# Autodesk Inventor assembly: x_iddler
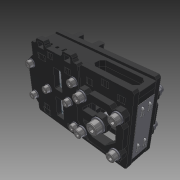
[picture p0: Inventor's stored thumbnail of the model, 180x180]
Saved by Autodesk Inventor 2014 (Build 180170000, 170)
## iProperties
Created: 2014-04-03
Part Number: x_iddler
Document SubType Name: Assembly
Designer: buben
Author: buben
## Documents named in this file (31)
- C:\Users\buben\Documents\GitHub\bacon\inventor files\assemblies\x_iddler.iam
- C:\Users\buben\Documents\GitHub\bacon\inventor files\printer parts\x_iddler_back.ipt
- C:\Users\buben\Documents\GitHub\bacon\inventor files\printer parts\x_motor_smooth_rod_spacer.ipt
- C:\Users\buben\Documents\GitHub\bacon\inventor files\printer parts\x_iddler_wall_upper.ipt
- C:\Users\buben\Documents\GitHub\bacon\inventor files\printer parts\x_iddler_wall_lower.ipt
- C:\Users\buben\Documents\GitHub\bacon\inventor files\printer parts\x_iddler_upper_nut_stop.ipt
- C:\Users\buben\Documents\GitHub\bacon\inventor files\printer parts\x_motor_middle.ipt
- C:\Users\buben\Documents\GitHub\bacon\inventor files\3rd party components\linear_bearing_8\Imported Components\LU8MM\LU8MM.iam
- C:\Users\buben\Documents\GitHub\bacon\inventor files\printer parts\x_motor_top.ipt
- C:\Users\buben\Documents\GitHub\bacon\inventor files\printer parts\x_motor_lower_nut_stop.ipt
- C:\Users\buben\Documents\GitHub\bacon\inventor files\utils\washer_m4.ipt
- C:\Users\buben\Documents\Inventor\Content Center Files\R2014\en-US\ISO 4762(2)\ISO 4762 - M4 x 20ISO.ipt
- C:\Users\buben\Documents\Inventor\Content Center Files\R2014\en-US\ISO 7040\ISO 7040 - M4.ipt
- C:\Users\buben\Documents\Inventor\Content Center Files\R2014\en-US\CSN EN 24032\ISO 4032 - M5CSN EN.ipt
- C:\Users\buben\Documents\GitHub\bacon\inventor files\utils\washer_m5.ipt
- C:\Users\buben\Documents\Inventor\Content Center Files\R2014\en-US\ISO 4762(2)\ISO 4762 - M5 x 50ISO.ipt
- C:\Users\buben\Documents\Inventor\Content Center Files\R2014\en-US\ISO 7040\ISO 7040 - M5.ipt
- C:\Users\buben\Documents\GitHub\bacon\inventor files\printer parts\x_iddler_c_mount.ipt
- C:\Users\buben\Documents\GitHub\bacon\inventor files\printer parts\x_iddler_belt_bearing_mount.ipt
- C:\Users\buben\Documents\GitHub\bacon\inventor files\utils\washer_m6.ipt
- C:\Users\buben\Documents\Inventor\Content Center Files\R2014\en-US\ISO 4762(2)\ISO 4762 - M6 x 60ISO.ipt
- C:\Users\buben\Documents\Inventor\Content Center Files\R2014\en-US\ISO 7040\ISO 7040 - M6.ipt
- C:\Users\buben\Documents\GitHub\bacon\inventor files\utils\washer_m8.ipt
- C:\Users\buben\Documents\Inventor\Content Center Files\R2014\en-US\ISO 7040\ISO 7040 - M8.ipt
- C:\Users\buben\Documents\Inventor\Content Center Files\R2014\en-US\ISO 4762(2)\ISO 4762 - M8 x 65ISO.ipt
- C:\Users\buben\Documents\GitHub\bacon\inventor files\3rd party components\bearing_608\Imported Components\608RS\608RS.ipt
- C:\Users\buben\Documents\GitHub\bacon\inventor files\utils\belt_guide.ipt
- C:\Users\buben\Documents\GitHub\bacon\inventor files\utils\bearing_spacer_1.ipt
- C:\Users\buben\Documents\GitHub\bacon\inventor files\utils\bearing_spacer_2.ipt
- C:\Users\buben\Documents\GitHub\bacon\inventor files\printer parts\x_iddler_right_cap.ipt
- C:\Users\buben\Documents\GitHub\bacon\inventor files\utils\x_iddler_cap_zip_tie.ipt
## Components (80 placed, 30 different names)
1. x_iddler_back:1 — Mate:1, Mate:2, Mate:3, Mate:4, Mate:5, Mate:6, Mate:7, Mate:8, Mate:9, Mate:10, Mate:11, Mate:12, Mate:13, Mate:14, Mate:15, Mate:16, Mate:17, Mate:18, Mate:56, Mate:57, Mate:58, Mate:59, Mate:60, Mate:61, Mate:89, Mate:90, Mate:91, Mate:140
2. x_motor_smooth_rod_spacer:1 — Mate:4, Mate:7, Mate:8
3. x_motor_smooth_rod_spacer:2 — Mate:5, Mate:6, Mate:9
4. x_iddler_wall_upper:1 — Mate:10, Mate:11, Mate:12, Mate:19, Mate:21, Mate:27, Mate:28, Mate:44, Mate:45, Mate:141
5. x_iddler_wall_lower:1 — Mate:13, Mate:14, Mate:15, Mate:20, Flush:1, Mate:30, Mate:31, Mate:32, Mate:33, Mate:34, Mate:35, Mate:47, Mate:48
6. x_iddler_upper_nut_stop:1 — Mate:16, Mate:17, Mate:18, Mate:46, Mate:86, Mate:87, Mate:88
7. x_motor_middle:1 — Mate:19, Mate:20, Mate:21, Mate:22, Mate:23, Mate:24, Mate:26
8. LU8MM:1 [sub-assembly] — Mate:22, Mate:23, Mate:24, Mate:25, Mate:29
9. LU8MM:2 [sub-assembly] — Mate:25, Mate:26
10. x_motor_top:1 — Mate:27, Mate:28, Mate:29, Mate:50, Mate:51, Mate:52, Mate:53, Mate:54, Mate:55, Mate:62, Mate:63, Mate:64, Mate:65, Mate:66, Mate:67
11. x_motor_lower_nut_stop:1 — Flush:1, Mate:30, Mate:31, Mate:36, Mate:38, Mate:49
12. CSN 02 1702 B B 4,3:1 — Mate:36, Mate:37, Mate:40
13. CSN 02 1702 B B 4,3:2 — Mate:38, Mate:39, Mate:42
14. CSN 02 1702 B B 4,3:3 — Mate:33, Mate:34, Insert:2
15. CSN 02 1702 B B 4,3:4 — Mate:32, Mate:35, Insert:1
16. ISO 4762 M4 x 20:1 — Insert:1, Mate:37, Mate:41
17. ISO 4762 M4 x 20:2 — Insert:2, Mate:39, Mate:43
18. DIN EN ISO 7040 M4:1 — Mate:40, Mate:41
19. DIN EN ISO 7040 M4:2 — Mate:42, Mate:43
20. CSN EN 24032 M5:1 — Mate:44, Mate:45, Mate:46
21. CSN EN 24032 M5:2 — Mate:47, Mate:48, Mate:49
22. CSN 02 1702 B B 5,3:1 — Mate:58, Mate:72, Mate:82
23. CSN 02 1702 B B 5,3:2 — Mate:57, Mate:70, Mate:78
24. CSN 02 1702 B B 5,3:3 — Mate:60, Mate:68, Mate:76
25. CSN 02 1702 B B 5,3:4 — Mate:61, Mate:69, Mate:80
26. CSN 02 1702 B B 5,3:5 — Mate:59, Mate:73, Mate:84
27. CSN 02 1702 B B 5,3:6 — Mate:56, Mate:71, Mate:74
28. CSN 02 1702 B B 5,3:7 — Mate:54, Mate:66, Insert:7
29. CSN 02 1702 B B 5,3:8 — Mate:51, Mate:63, Insert:3
30. CSN 02 1702 B B 5,3:9 — Mate:50, Mate:62, Insert:4
31. CSN 02 1702 B B 5,3:10 — Mate:55, Mate:67, Insert:6
32. CSN 02 1702 B B 5,3:11 — Mate:53, Mate:65, Insert:8
33. CSN 02 1702 B B 5,3:12 — Mate:52, Mate:64, Insert:5
34. ISO 4762 M5 x 50:1 — Insert:3, Mate:68, Mate:77
35. ISO 4762 M5 x 50:2 — Insert:4, Mate:69, Mate:81
36. ISO 4762 M5 x 50:3 — Insert:5, Mate:70, Mate:79
37. ISO 4762 M5 x 50:4 — Insert:6, Mate:71, Mate:75
38. ISO 4762 M5 x 50:5 — Insert:7, Mate:72, Mate:83
39. ISO 4762 M5 x 50:6 — Insert:8, Mate:73, Mate:85
40. DIN EN ISO 7040 M5:1 — Mate:78, Mate:79
41. DIN EN ISO 7040 M5:2 — Mate:80, Mate:81
42. DIN EN ISO 7040 M5:3 — Mate:84, Mate:85
43. DIN EN ISO 7040 M5:4 — Mate:82, Mate:83
44. DIN EN ISO 7040 M5:5 — Mate:76, Mate:77
45. DIN EN ISO 7040 M5:6 — Mate:74, Mate:75
46. x_iddler_c_mount:1 — Mate:86, Mate:87, Mate:88, Mate:92, Mate:93, Mate:94
47. x_iddler_belt_bearing_mount:1 — Mate:89, Mate:90, Mate:91, Mate:103, Mate:105, Mate:107, Mate:109, Mate:121, Mate:122, Mate:125, Mate:126
48. x_iddler_belt_bearing_mount:2 — Mate:92, Mate:93, Mate:94, Mate:95, Mate:96, Mate:97, Mate:98, Mate:99, Mate:100, Mate:101, Mate:102, Mate:119, Mate:120, Mate:123, Mate:124
49. CSN 02 1702 B B 6,4:1 — Mate:105, Mate:106, Mate:115
50. CSN 02 1702 B B 6,4:2 — Mate:101, Mate:102, Insert:10
51. CSN 02 1702 B B 6,4:3 — Mate:103, Mate:104, Mate:117
52. CSN 02 1702 B B 6,4:4 — Mate:107, Mate:108, Mate:111
53. CSN 02 1702 B B 6,4:5 — Mate:109, Mate:110, Mate:113
54. CSN 02 1702 B B 6,4:6 — Mate:99, Mate:100, Insert:11
55. CSN 02 1702 B B 6,4:7 — Mate:97, Mate:98, Insert:12
56. CSN 02 1702 B B 6,4:8 — Mate:95, Mate:96, Insert:9
57. ISO 4762 M6 x 60:3 — Insert:9, Mate:110, Mate:114
58. ISO 4762 M6 x 60:4 — Insert:10, Mate:108, Mate:112, Mate:144, Mate:145
59. ISO 4762 M6 x 60:2 — Insert:11, Mate:104, Mate:118, Tangent:1, Mate:142, Mate:143
60. ISO 4762 M6 x 60:1 — Insert:12, Mate:106, Mate:116
61. DIN EN ISO 7040 M6:1 — Mate:115, Mate:116
62. DIN EN ISO 7040 M6:2 — Mate:111, Mate:112
63. DIN EN ISO 7040 M6:3 — Mate:113, Mate:114
64. DIN EN ISO 7040 M6:4 — Mate:117, Mate:118
65. CSN 02 1702 B B 8,4:1 — Mate:119, Mate:120, Insert:13
66. CSN 02 1702 B B 8,4:2 — Mate:121, Mate:122, Mate:127
67. CSN 02 1702 B B 8,4:3 — Mate:123, Mate:124
68. CSN 02 1702 B B 8,4:4 — Mate:125, Mate:126, Mate:136
69. ISO 4762 M8 x 65:1 — Insert:13, Mate:128, Mate:139
70. DIN EN ISO 7040 M8:1 — Mate:127, Mate:128
71. 608RS:1 — Mate:129, Mate:130, Mate:133, Mate:134, Mate:135, Mate:137, Mate:138
72. belt_guide:1 — Mate:129, Mate:130, Mate:131, Mate:132
73. belt_guide:2 — Mate:131, Mate:132, Mate:133
74. bearing_spacer_1:1 — Mate:134, Mate:135, Mate:136
75. bearing_spacer_2:1 — Mate:137, Mate:138, Mate:139
76. x_iddler_right_cap:1 — Mate:140, Mate:141, Tangent:1, Angle:1, Angle:2, Angle:3, Angle:4, Tangent:2, Tangent:3, Tangent:4, Tangent:5
77. x_iddler_cap_zip_tie:1 — Mate:142, Angle:3, Tangent:3
78. x_iddler_cap_zip_tie:2 — Mate:143, Angle:1, Tangent:4
79. x_iddler_cap_zip_tie:3 — Mate:144, Angle:4, Tangent:2
80. x_iddler_cap_zip_tie:4 — Mate:145, Angle:2, Tangent:5
## Relationships (168: Mate 145, Insert 13, Tangent 5, Angle 4, Flush 1)
- Mate:1: x_iddler_back:1
- Mate:2: x_iddler_back:1
- Mate:3: x_iddler_back:1
- Mate:4: x_iddler_back:1 ↔ x_motor_smooth_rod_spacer:1
- Mate:5: x_iddler_back:1 ↔ x_motor_smooth_rod_spacer:2
- Mate:6: x_iddler_back:1 ↔ x_motor_smooth_rod_spacer:2
- Mate:7: x_iddler_back:1 ↔ x_motor_smooth_rod_spacer:1
- Mate:8: x_iddler_back:1 ↔ x_motor_smooth_rod_spacer:1
- Mate:9: x_iddler_back:1 ↔ x_motor_smooth_rod_spacer:2
- Mate:10: x_iddler_back:1 ↔ x_iddler_wall_upper:1
- Mate:11: x_iddler_back:1 ↔ x_iddler_wall_upper:1
- Mate:12: x_iddler_back:1 ↔ x_iddler_wall_upper:1
- Mate:13: x_iddler_back:1 ↔ x_iddler_wall_lower:1
- Mate:14: x_iddler_back:1 ↔ x_iddler_wall_lower:1
- Mate:15: x_iddler_back:1 ↔ x_iddler_wall_lower:1
- Mate:16: x_iddler_back:1 ↔ x_iddler_upper_nut_stop:1
- Mate:17: x_iddler_back:1 ↔ x_iddler_upper_nut_stop:1
- Mate:18: x_iddler_back:1 ↔ x_iddler_upper_nut_stop:1
- Mate:19: x_iddler_wall_upper:1 ↔ x_motor_middle:1
- Mate:20: x_iddler_wall_lower:1 ↔ x_motor_middle:1
- Mate:21: x_iddler_wall_upper:1 ↔ x_motor_middle:1
- Mate:22 (7.5 mm): x_motor_middle:1 ↔ LU8MM:1
- Mate:23 (7.5 mm): x_motor_middle:1 ↔ LU8MM:1
- Mate:24 (0.5 mm): x_motor_middle:1 ↔ LU8MM:1
- Mate:25: LU8MM:1 ↔ LU8MM:2
- Mate:26 (0.5 mm): x_motor_middle:1 ↔ LU8MM:2
- Mate:27: x_iddler_wall_upper:1 ↔ x_motor_top:1
- Mate:28: x_iddler_wall_upper:1 ↔ x_motor_top:1
- Mate:29 (7.5 mm): LU8MM:1 ↔ x_motor_top:1
- Flush:1: x_iddler_wall_lower:1 ↔ x_motor_lower_nut_stop:1
- Mate:30: x_iddler_wall_lower:1 ↔ x_motor_lower_nut_stop:1
- Mate:31: x_iddler_wall_lower:1 ↔ x_motor_lower_nut_stop:1
- Mate:32: x_iddler_wall_lower:1 ↔ CSN 02 1702 B B 4,3:4
- Mate:33: x_iddler_wall_lower:1 ↔ CSN 02 1702 B B 4,3:3
- Mate:34: x_iddler_wall_lower:1 ↔ CSN 02 1702 B B 4,3:3
- Mate:35: x_iddler_wall_lower:1 ↔ CSN 02 1702 B B 4,3:4
- Insert:1: CSN 02 1702 B B 4,3:4 ↔ ISO 4762 M4 x 20:1
- Insert:2: CSN 02 1702 B B 4,3:3 ↔ ISO 4762 M4 x 20:2
- Mate:36: x_motor_lower_nut_stop:1 ↔ CSN 02 1702 B B 4,3:1
- Mate:37: CSN 02 1702 B B 4,3:1 ↔ ISO 4762 M4 x 20:1
- Mate:38: x_motor_lower_nut_stop:1 ↔ CSN 02 1702 B B 4,3:2
- Mate:39: CSN 02 1702 B B 4,3:2 ↔ ISO 4762 M4 x 20:2
- Mate:40: CSN 02 1702 B B 4,3:1 ↔ DIN EN ISO 7040 M4:1
- Mate:41: ISO 4762 M4 x 20:1 ↔ DIN EN ISO 7040 M4:1
- Mate:42: CSN 02 1702 B B 4,3:2 ↔ DIN EN ISO 7040 M4:2
- Mate:43: ISO 4762 M4 x 20:2 ↔ DIN EN ISO 7040 M4:2
- Mate:44: x_iddler_wall_upper:1 ↔ CSN EN 24032 M5:1
- Mate:45: x_iddler_wall_upper:1 ↔ CSN EN 24032 M5:1
- Mate:46: x_iddler_upper_nut_stop:1 ↔ CSN EN 24032 M5:1
- Mate:47: x_iddler_wall_lower:1 ↔ CSN EN 24032 M5:2
- Mate:48: x_iddler_wall_lower:1 ↔ CSN EN 24032 M5:2
- Mate:49: x_motor_lower_nut_stop:1 ↔ CSN EN 24032 M5:2
- Mate:50: x_motor_top:1 ↔ CSN 02 1702 B B 5,3:9
- Mate:51: x_motor_top:1 ↔ CSN 02 1702 B B 5,3:8
- Mate:52: x_motor_top:1 ↔ CSN 02 1702 B B 5,3:12
- Mate:53: x_motor_top:1 ↔ CSN 02 1702 B B 5,3:11
- Mate:54: x_motor_top:1 ↔ CSN 02 1702 B B 5,3:7
- Mate:55: x_motor_top:1 ↔ CSN 02 1702 B B 5,3:10
- Mate:56: x_iddler_back:1 ↔ CSN 02 1702 B B 5,3:6
- Mate:57: x_iddler_back:1 ↔ CSN 02 1702 B B 5,3:2
- Mate:58: x_iddler_back:1 ↔ CSN 02 1702 B B 5,3:1
- Mate:59: x_iddler_back:1 ↔ CSN 02 1702 B B 5,3:5
- Mate:60: x_iddler_back:1 ↔ CSN 02 1702 B B 5,3:3
- Mate:61: x_iddler_back:1 ↔ CSN 02 1702 B B 5,3:4
- Mate:62: x_motor_top:1 ↔ CSN 02 1702 B B 5,3:9
- Mate:63: x_motor_top:1 ↔ CSN 02 1702 B B 5,3:8
- Mate:64: x_motor_top:1 ↔ CSN 02 1702 B B 5,3:12
- Mate:65: x_motor_top:1 ↔ CSN 02 1702 B B 5,3:11
- Mate:66: x_motor_top:1 ↔ CSN 02 1702 B B 5,3:7
- Mate:67: x_motor_top:1 ↔ CSN 02 1702 B B 5,3:10
- Insert:3: CSN 02 1702 B B 5,3:8 ↔ ISO 4762 M5 x 50:1
- Insert:4: CSN 02 1702 B B 5,3:9 ↔ ISO 4762 M5 x 50:2
- Insert:5: CSN 02 1702 B B 5,3:12 ↔ ISO 4762 M5 x 50:3
- Insert:6: CSN 02 1702 B B 5,3:10 ↔ ISO 4762 M5 x 50:4
- Insert:7: CSN 02 1702 B B 5,3:7 ↔ ISO 4762 M5 x 50:5
- Insert:8: CSN 02 1702 B B 5,3:11 ↔ ISO 4762 M5 x 50:6
- Mate:68: CSN 02 1702 B B 5,3:3 ↔ ISO 4762 M5 x 50:1
- Mate:69: CSN 02 1702 B B 5,3:4 ↔ ISO 4762 M5 x 50:2
- Mate:70: CSN 02 1702 B B 5,3:2 ↔ ISO 4762 M5 x 50:3
- Mate:71: CSN 02 1702 B B 5,3:6 ↔ ISO 4762 M5 x 50:4
- Mate:72: CSN 02 1702 B B 5,3:1 ↔ ISO 4762 M5 x 50:5
- Mate:73: CSN 02 1702 B B 5,3:5 ↔ ISO 4762 M5 x 50:6
- Mate:74: CSN 02 1702 B B 5,3:6 ↔ DIN EN ISO 7040 M5:6
- Mate:75: ISO 4762 M5 x 50:4 ↔ DIN EN ISO 7040 M5:6
- Mate:76: CSN 02 1702 B B 5,3:3 ↔ DIN EN ISO 7040 M5:5
- Mate:77: ISO 4762 M5 x 50:1 ↔ DIN EN ISO 7040 M5:5
- Mate:78: CSN 02 1702 B B 5,3:2 ↔ DIN EN ISO 7040 M5:1
- Mate:79: ISO 4762 M5 x 50:3 ↔ DIN EN ISO 7040 M5:1
- Mate:80: CSN 02 1702 B B 5,3:4 ↔ DIN EN ISO 7040 M5:2
- Mate:81: ISO 4762 M5 x 50:2 ↔ DIN EN ISO 7040 M5:2
- Mate:82: CSN 02 1702 B B 5,3:1 ↔ DIN EN ISO 7040 M5:4
- Mate:83: ISO 4762 M5 x 50:5 ↔ DIN EN ISO 7040 M5:4
- Mate:84: CSN 02 1702 B B 5,3:5 ↔ DIN EN ISO 7040 M5:3
- Mate:85: ISO 4762 M5 x 50:6 ↔ DIN EN ISO 7040 M5:3
- Mate:86: x_iddler_upper_nut_stop:1 ↔ x_iddler_c_mount:1
- Mate:87: x_iddler_upper_nut_stop:1 ↔ x_iddler_c_mount:1
- Mate:88: x_iddler_upper_nut_stop:1 ↔ x_iddler_c_mount:1
- Mate:89: x_iddler_back:1 ↔ x_iddler_belt_bearing_mount:1
- Mate:90: x_iddler_back:1 ↔ x_iddler_belt_bearing_mount:1
- Mate:91: x_iddler_back:1 ↔ x_iddler_belt_bearing_mount:1
- Mate:92: x_iddler_c_mount:1 ↔ x_iddler_belt_bearing_mount:2
- Mate:93: x_iddler_c_mount:1 ↔ x_iddler_belt_bearing_mount:2
- Mate:94: x_iddler_c_mount:1 ↔ x_iddler_belt_bearing_mount:2
- Mate:95: x_iddler_belt_bearing_mount:2 ↔ CSN 02 1702 B B 6,4:8
- Mate:96: x_iddler_belt_bearing_mount:2 ↔ CSN 02 1702 B B 6,4:8
- Mate:97: x_iddler_belt_bearing_mount:2 ↔ CSN 02 1702 B B 6,4:7
- Mate:98: x_iddler_belt_bearing_mount:2 ↔ CSN 02 1702 B B 6,4:7
- Mate:99: x_iddler_belt_bearing_mount:2 ↔ CSN 02 1702 B B 6,4:6
- Mate:100: x_iddler_belt_bearing_mount:2 ↔ CSN 02 1702 B B 6,4:6
- Mate:101: x_iddler_belt_bearing_mount:2 ↔ CSN 02 1702 B B 6,4:2
- Mate:102: x_iddler_belt_bearing_mount:2 ↔ CSN 02 1702 B B 6,4:2
- Insert:9: CSN 02 1702 B B 6,4:8 ↔ ISO 4762 M6 x 60:3
- Insert:10: CSN 02 1702 B B 6,4:2 ↔ ISO 4762 M6 x 60:4
- Insert:11: CSN 02 1702 B B 6,4:6 ↔ ISO 4762 M6 x 60:2
- Insert:12: CSN 02 1702 B B 6,4:7 ↔ ISO 4762 M6 x 60:1
- Mate:103: x_iddler_belt_bearing_mount:1 ↔ CSN 02 1702 B B 6,4:3
- Mate:104: CSN 02 1702 B B 6,4:3 ↔ ISO 4762 M6 x 60:2
- Mate:105: x_iddler_belt_bearing_mount:1 ↔ CSN 02 1702 B B 6,4:1
- Mate:106: CSN 02 1702 B B 6,4:1 ↔ ISO 4762 M6 x 60:1
- Mate:107: x_iddler_belt_bearing_mount:1 ↔ CSN 02 1702 B B 6,4:4
- Mate:108: CSN 02 1702 B B 6,4:4 ↔ ISO 4762 M6 x 60:4
- Mate:109: x_iddler_belt_bearing_mount:1 ↔ CSN 02 1702 B B 6,4:5
- Mate:110: CSN 02 1702 B B 6,4:5 ↔ ISO 4762 M6 x 60:3
- Mate:111: CSN 02 1702 B B 6,4:4 ↔ DIN EN ISO 7040 M6:2
- Mate:112: ISO 4762 M6 x 60:4 ↔ DIN EN ISO 7040 M6:2
- Mate:113: CSN 02 1702 B B 6,4:5 ↔ DIN EN ISO 7040 M6:3
- Mate:114: ISO 4762 M6 x 60:3 ↔ DIN EN ISO 7040 M6:3
- Mate:115: CSN 02 1702 B B 6,4:1 ↔ DIN EN ISO 7040 M6:1
- Mate:116: ISO 4762 M6 x 60:1 ↔ DIN EN ISO 7040 M6:1
- Mate:117: CSN 02 1702 B B 6,4:3 ↔ DIN EN ISO 7040 M6:4
- Mate:118: ISO 4762 M6 x 60:2 ↔ DIN EN ISO 7040 M6:4
- Mate:119: x_iddler_belt_bearing_mount:2 ↔ CSN 02 1702 B B 8,4:1
- Mate:120: x_iddler_belt_bearing_mount:2 ↔ CSN 02 1702 B B 8,4:1
- Mate:121: x_iddler_belt_bearing_mount:1 ↔ CSN 02 1702 B B 8,4:2
- Mate:122: x_iddler_belt_bearing_mount:1 ↔ CSN 02 1702 B B 8,4:2
- Mate:123: x_iddler_belt_bearing_mount:2 ↔ CSN 02 1702 B B 8,4:3
- Mate:124: x_iddler_belt_bearing_mount:2 ↔ CSN 02 1702 B B 8,4:3
- Mate:125: x_iddler_belt_bearing_mount:1 ↔ CSN 02 1702 B B 8,4:4
- Mate:126: x_iddler_belt_bearing_mount:1 ↔ CSN 02 1702 B B 8,4:4
- Insert:13: CSN 02 1702 B B 8,4:1 ↔ ISO 4762 M8 x 65:1
- Mate:127: CSN 02 1702 B B 8,4:2 ↔ DIN EN ISO 7040 M8:1
- Mate:128: ISO 4762 M8 x 65:1 ↔ DIN EN ISO 7040 M8:1
- Mate:129: 608RS:1 ↔ belt_guide:1
- Mate:130: 608RS:1 ↔ belt_guide:1
- Mate:131: belt_guide:1 ↔ belt_guide:2
- Mate:132: belt_guide:1 ↔ belt_guide:2
- Mate:133: 608RS:1 ↔ belt_guide:2
- Mate:134: 608RS:1 ↔ bearing_spacer_1:1
- Mate:135: 608RS:1 ↔ bearing_spacer_1:1
- Mate:136: CSN 02 1702 B B 8,4:4 ↔ bearing_spacer_1:1
- Mate:137: 608RS:1 ↔ bearing_spacer_2:1
- Mate:138: 608RS:1 ↔ bearing_spacer_2:1
- Mate:139: ISO 4762 M8 x 65:1 ↔ bearing_spacer_2:1
- Mate:140: x_iddler_back:1 ↔ x_iddler_right_cap:1
- Mate:141: x_iddler_wall_upper:1 ↔ x_iddler_right_cap:1
- Tangent:1: ISO 4762 M6 x 60:2 ↔ x_iddler_right_cap:1
- Mate:142: ISO 4762 M6 x 60:2 ↔ x_iddler_cap_zip_tie:1
- Mate:143: ISO 4762 M6 x 60:2 ↔ x_iddler_cap_zip_tie:2
- Mate:144: ISO 4762 M6 x 60:4 ↔ x_iddler_cap_zip_tie:3
- Mate:145: ISO 4762 M6 x 60:4 ↔ x_iddler_cap_zip_tie:4
- Angle:1 (180 deg): x_iddler_right_cap:1 ↔ x_iddler_cap_zip_tie:2
- Angle:2 (180 deg): x_iddler_right_cap:1 ↔ x_iddler_cap_zip_tie:4
- Angle:3 (180 deg): x_iddler_right_cap:1 ↔ x_iddler_cap_zip_tie:1
- Angle:4 (180 deg): x_iddler_right_cap:1 ↔ x_iddler_cap_zip_tie:3
- Tangent:2: x_iddler_right_cap:1 ↔ x_iddler_cap_zip_tie:3
- Tangent:3: x_iddler_right_cap:1 ↔ x_iddler_cap_zip_tie:1
- Tangent:4: x_iddler_right_cap:1 ↔ x_iddler_cap_zip_tie:2
- Tangent:5: x_iddler_right_cap:1 ↔ x_iddler_cap_zip_tie:4
